# Autodesk Inventor assembly: Delta Manipulator
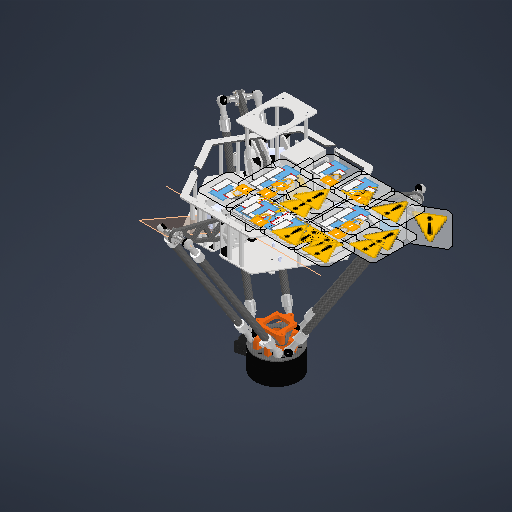
[picture p0: Inventor's stored thumbnail of the model, 512x512]
Saved by Autodesk Inventor 2026.3 (Build 303398000, 398)
## iProperties
Created: 2025-09-05
Part Number: Delta Manipulator
Document SubType Name: Assembly
Designer: Xiao
Mass: 3353.65 g
Surface Area: 7565.1 cm^2
Volume: 948.398 cm^3
Density: 3.53611 g/cm^3
Author: Xiao
## Documents named in this file (12)
- C:\Users\陈嘉瑞\Desktop\3-DoF\修改云台画图\Delta Manipulator.iam
- C:\Users\陈嘉瑞\Desktop\3-DoF\Manipulator\Link2.iam
- C:\Users\陈嘉瑞\Desktop\3-DoF\Manipulator\动平台.iam
- C:\Users\陈嘉瑞\Desktop\3-DoF\Manipulator\无人机组件.iam
- C:\Users\陈嘉瑞\Desktop\3-DoF\Manipulator\摇臂.iam
- C:\Users\陈嘉瑞\Desktop\3-DoF\Manipulator\三角角码.ipt
- C:\Users\陈嘉瑞\Desktop\3-DoF\Manipulator\分电板\RM_ESC_Center_Board2\RM_ESC_Center_Board2\RM_ESC_Center_Board2.iam
- C:\Users\陈嘉瑞\Desktop\3-DoF\Manipulator\M2.5x6尼龙柱.ipt
- C:\Users\陈嘉瑞\Desktop\3-DoF\Manipulator\M3-60 六角铝柱.ipt
- C:\Users\陈嘉瑞\Desktop\3-DoF\Manipulator\M3-20 六角铝柱.ipt
- F:\Control System Lab\Delta Aerial manipulator\Drone\zd-680-carbon-fiber-frame-1.snapshot.1\main assambly STEP\main assambly STEP\main assambly STEP.iam
- C:\Users\陈嘉瑞\Desktop\3-DoF\修改云台画图\云台基座.iam
## Components (77 placed, 11 different names)
1. 动平台:1 [sub-assembly] — 球:3, 球:4, 球:5, 球:6, 球:7, 球:8
2. Link2:1 [sub-assembly] — 球:8, 球:10
3. Link2:2 [sub-assembly] — 球:7, 球:9
4. Link2:3 [sub-assembly] — 球:3, 球:11
5. Link2:4 [sub-assembly] — 球:4, 球:12
6. Link2:5 [sub-assembly] — 球:5, 球:14
7. Link2:6 [sub-assembly] — 球:6, 球:13
8. 无人机组件:1 [sub-assembly] — 配合:3
9. 摇臂:1 [sub-assembly] — 球:9, 球:10, 配合:5, 配合:7, 配合:11, 配合:12, 配合:16
10. 摇臂:2 [sub-assembly] — 球:11, 球:12, 配合:4, 配合:17, 配合:18
11. 摇臂:3 [sub-assembly] — 旋转:3, 球:13, 球:14, 配合:6, 配合:14, 配合:15
12. 云台基座:1 [sub-assembly] — 表面齐平:2, 表面齐平:3, 配合:3, 旋转:3, 插入:3, 插入:5, 插入:6, 插入:7, 插入:11, 插入:12, 插入:13, 插入:14, 插入:17, 插入:18, 插入:19, 插入:20, 插入:21, 插入:22, 插入:23, 插入:24, 插入:25, 插入:26, 插入:27, 插入:28, 插入:29, 插入:30, 插入:31, 插入:32, 插入:33, 插入:34, 插入:35, 插入:36, 插入:39, 插入:40, 插入:41, 插入:42, 插入:43, 插入:44, 插入:45, 插入:46, 插入:47, 插入:48, 插入:49, 插入:50, 插入:51, 配合:4, 配合:5, 配合:6, 配合:11, 配合:12, 配合:14, 配合:15, 配合:16, 配合:17, 配合:18
13. RM_ESC_Center_Board2:1 [sub-assembly] — 插入:37, 插入:38
14. M2.5x6尼龙柱:1 — 插入:33
15. M2.5x6尼龙柱:2 — 插入:35, 插入:38
16. M2.5x6尼龙柱:3 — 插入:34
17. M2.5x6尼龙柱:4 — 插入:36, 插入:37
18. M3-20 六角铝柱:1 — 插入:44, 插入:52
19. M3-20 六角铝柱:2 — 插入:45, 插入:53
20. M3-20 六角铝柱:3 — 插入:51
21. M3-20 六角铝柱:4 — 插入:50
22. M3-20 六角铝柱:5 — 插入:46
23. M3-20 六角铝柱:6 — 插入:47
24. M3-20 六角铝柱:7 — 插入:48
25. M3-20 六角铝柱:8 — 插入:49
26. main assambly STEP:1 [sub-assembly] — 插入:52, 插入:53
27. 三角角码:1 — 插入:6, 插入:7
28. 三角角码:2 — 插入:13, 插入:14
29. 三角角码:3 — 插入:3, 插入:5
30. 三角角码:4 — 插入:11, 插入:12
31. 三角角码:5 — 插入:19, 插入:20
32. 三角角码:6 — 插入:23, 插入:24
33. 三角角码:7 — 插入:17, 插入:18
34. 三角角码:8 — 插入:21, 插入:22
35. 三角角码:9 — 插入:25, 插入:27
36. 三角角码:10 — 插入:26, 插入:28
37. 三角角码:11 — 插入:29, 插入:31
38. 三角角码:12 — 插入:30, 插入:32
39. 三角角码:13
40. 三角角码:14
41. 三角角码:15
42. 三角角码:16
43. 三角角码:17
44. 三角角码:18
45. 三角角码:19
46. 三角角码:20
47. 三角角码:21
48. 三角角码:22
49. 三角角码:23
50. 三角角码:24
51. 三角角码:25
52. 三角角码:26
53. 三角角码:27
54. 三角角码:28
55. 三角角码:29
56. 三角角码:30
57. 三角角码:31
58. 三角角码:32
59. 三角角码:33
60. 三角角码:34
61. 三角角码:35
62. 三角角码:36
63. M3-60 六角铝柱:2 — 插入:41
64. M3-60 六角铝柱:1 — 插入:40
65. M3-60 六角铝柱:4 — 插入:43
66. M3-60 六角铝柱:3 — 插入:42
67. M3-60 六角铝柱:5 — 插入:39
68. M3-60 六角铝柱:6
69. M3-60 六角铝柱:7
70. M3-60 六角铝柱:8
71. M3-60 六角铝柱:9
72. M3-60 六角铝柱:10
73. M3-60 六角铝柱:11
74. M3-60 六角铝柱:12
75. M3-60 六角铝柱:13
76. M3-60 六角铝柱:14
77. M3-60 六角铝柱:15
## Component patterns: (3 elements, first: 三角角码:1 + 三角角码:2 + 三角角码:3 + 三角角码:4 + 三角角码:5 + 三角角码:6 + 三角角码:7 + 三角角码:8 + 三角角码:9 + 三角角码:10 + 三角角码:11 + 三角角码:12), (3 elements, first: M3-60 六角铝柱:2 + M3-60 六角铝柱:1 + M3-60 六角铝柱:4 + M3-60 六角铝柱:3 + M3-60 六角铝柱:5)
## Relationships (76: Insert 45, Mate 14, BallJoint 12, RevoluteJoint 3, Flush 2)
- 球:3 [BallJoint]: 动平台:1 ↔ Link2:3
- 球:4 [BallJoint]: 动平台:1 ↔ Link2:4
- 球:5 [BallJoint]: 动平台:1 ↔ Link2:5
- 球:6 [BallJoint]: 动平台:1 ↔ Link2:6
- 球:7 [BallJoint]: 动平台:1 ↔ Link2:2
- 球:8 [BallJoint]: 动平台:1 ↔ Link2:1
- 球:9 [BallJoint]: Link2:2 ↔ 摇臂:1
- 球:10 [BallJoint]: Link2:1 ↔ 摇臂:1
- 球:11 [BallJoint]: Link2:3 ↔ 摇臂:2
- 球:12 [BallJoint]: Link2:4 ↔ 摇臂:2
- 表面齐平:2 [Flush]: 云台基座:1
- 表面齐平:3 [Flush]: 云台基座:1
- 配合:3 [Mate] (59.5 mm): 无人机组件:1 ↔ 云台基座:1
- [RevoluteJoint]: 摇臂:1 ↔ 云台基座:1
- [RevoluteJoint]: 摇臂:2 ↔ 云台基座:1
- 旋转:3 [RevoluteJoint]: 摇臂:3 ↔ 云台基座:1
- 球:13 [BallJoint]: Link2:6 ↔ 摇臂:3
- 球:14 [BallJoint]: Link2:5 ↔ 摇臂:3
- 插入:3 [Insert]: 云台基座:1 ↔ 三角角码:3
- 插入:5 [Insert]: 云台基座:1 ↔ 三角角码:3
- 插入:6 [Insert]: 云台基座:1 ↔ 三角角码:1
- 插入:7 [Insert]: 云台基座:1 ↔ 三角角码:1
- 插入:11 [Insert]: 云台基座:1 ↔ 三角角码:4
- 插入:12 [Insert]: 云台基座:1 ↔ 三角角码:4
- 插入:13 [Insert]: 云台基座:1 ↔ 三角角码:2
- 插入:14 [Insert]: 云台基座:1 ↔ 三角角码:2
- 插入:17 [Insert]: 云台基座:1 ↔ 三角角码:7
- 插入:18 [Insert]: 云台基座:1 ↔ 三角角码:7
- 插入:19 [Insert]: 云台基座:1 ↔ 三角角码:5
- 插入:20 [Insert]: 云台基座:1 ↔ 三角角码:5
- 插入:21 [Insert]: 云台基座:1 ↔ 三角角码:8
- 插入:22 [Insert]: 云台基座:1 ↔ 三角角码:8
- 插入:23 [Insert]: 云台基座:1 ↔ 三角角码:6
- 插入:24 [Insert]: 云台基座:1 ↔ 三角角码:6
- 插入:25 [Insert]: 云台基座:1 ↔ 三角角码:9
- 插入:26 [Insert]: 云台基座:1 ↔ 三角角码:10
- 插入:27 [Insert]: 云台基座:1 ↔ 三角角码:9
- 插入:28 [Insert]: 云台基座:1 ↔ 三角角码:10
- 插入:29 [Insert]: 云台基座:1 ↔ 三角角码:11
- 插入:30 [Insert]: 云台基座:1 ↔ 三角角码:12
- 插入:31 [Insert]: 云台基座:1 ↔ 三角角码:11
- 插入:32 [Insert]: 云台基座:1 ↔ 三角角码:12
- 插入:33 [Insert]: 云台基座:1 ↔ M2.5x6尼龙柱:1
- 插入:34 [Insert]: 云台基座:1 ↔ M2.5x6尼龙柱:3
- 插入:35 [Insert]: 云台基座:1 ↔ M2.5x6尼龙柱:2
- 插入:36 [Insert]: 云台基座:1 ↔ M2.5x6尼龙柱:4
- 插入:37 [Insert]: RM_ESC_Center_Board2:1 ↔ M2.5x6尼龙柱:4
- 插入:38 [Insert]: RM_ESC_Center_Board2:1 ↔ M2.5x6尼龙柱:2
- 插入:39 [Insert]: 云台基座:1 ↔ M3-60 六角铝柱:5
- 插入:40 [Insert]: 云台基座:1 ↔ M3-60 六角铝柱:1
- 插入:41 [Insert]: 云台基座:1 ↔ M3-60 六角铝柱:2
- 插入:42 [Insert]: 云台基座:1 ↔ M3-60 六角铝柱:3
- 插入:43 [Insert]: 云台基座:1 ↔ M3-60 六角铝柱:4
- 插入:44 [Insert]: 云台基座:1 ↔ M3-20 六角铝柱:1
- 插入:45 [Insert]: 云台基座:1 ↔ M3-20 六角铝柱:2
- 插入:46 [Insert]: 云台基座:1 ↔ M3-20 六角铝柱:5
- 插入:47 [Insert]: 云台基座:1 ↔ M3-20 六角铝柱:6
- 插入:48 [Insert]: 云台基座:1 ↔ M3-20 六角铝柱:7
- 插入:49 [Insert]: 云台基座:1 ↔ M3-20 六角铝柱:8
- 插入:50 [Insert]: 云台基座:1 ↔ M3-20 六角铝柱:4
- 插入:51 [Insert]: 云台基座:1 ↔ M3-20 六角铝柱:3
- 插入:52 [Insert]: M3-20 六角铝柱:1 ↔ main assambly STEP:1
- 插入:53 [Insert]: M3-20 六角铝柱:2 ↔ main assambly STEP:1
- 配合:4 [Mate]: 摇臂:2 ↔ 云台基座:1
- 配合:5 [Mate]: 摇臂:1 ↔ 云台基座:1
- 配合:6 [Mate]: 摇臂:3 ↔ 云台基座:1
- 配合:7 [Mate]: 摇臂:1
- 配合:9 [Mate]
- 配合:10 [Mate]
- 配合:11 [Mate]: 摇臂:1 ↔ 云台基座:1
- 配合:12 [Mate]: 摇臂:1 ↔ 云台基座:1
- 配合:14 [Mate]: 摇臂:3 ↔ 云台基座:1
- 配合:15 [Mate] (2 mm): 摇臂:3 ↔ 云台基座:1
- 配合:16 [Mate] (2 mm): 摇臂:1 ↔ 云台基座:1
- 配合:17 [Mate] (2 mm): 摇臂:2 ↔ 云台基座:1
- 配合:18 [Mate]: 摇臂:2 ↔ 云台基座:1
